# Autodesk Inventor assembly: arm j3 assembly
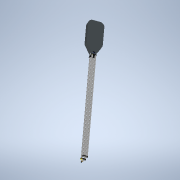
[picture p0: Inventor's stored thumbnail of the model, 180x180]
Saved by Autodesk Inventor 2020 (Build 240168000, 168)
## iProperties
Created: 2020-07-11
Part Number: arm j3 assembly
Document SubType Name: Assembly
Designer: Vikki
Mass: 3983.6 g
Surface Area: 16144.7 cm^2
Volume: 11217.3 cm^3
Density: 0.35513 g/cm^3
Author: Vikki
## Documents named in this file (5)
- E:\project inventor pro\flipkart grid models\articulated arm\arm j3 assembly.iam
- E:\project inventor pro\flipkart grid models\articulated arm\armj3.ipt
- E:\project inventor pro\flipkart grid models\articulated arm\joint.ipt
- E:\project inventor pro\flipkart grid models\articulated arm\joint 2.ipt
- E:\project inventor pro\flipkart grid models\articulated arm\2020 aluminum ext.ipt
## Components (4 placed, 4 different names)
1. armj3:1 — Mate:2, Flush:2, Flush:4
2. joint:1 — Mate:2, Flush:2, Mate:3, Flush:5, Flush:6
3. joint 2:1 — Flush:4
4. 2020 aluminum ext:1 — Mate:3, Flush:5, Flush:6
## Relationships (6: Flush 4, Mate 2)
- Mate:2 (35 mm): armj3:1 ↔ joint:1
- Flush:2: armj3:1 ↔ joint:1
- Flush:4: armj3:1 ↔ joint 2:1
- Mate:3: joint:1 ↔ 2020 aluminum ext:1
- Flush:5: joint:1 ↔ 2020 aluminum ext:1
- Flush:6 (5 mm): joint:1 ↔ 2020 aluminum ext:1
